# Autodesk Inventor assembly: batterycart assemble
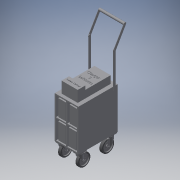
[picture p0: Inventor's stored thumbnail of the model, 180x180]
Saved by Autodesk Inventor 2019 (Build 230136000, 136)
## iProperties
Created: 2018-12-09
Part Number: batterycart assemble
Document SubType Name: Assembly
Designer: Tiberus
Author: Tiberus
## Documents named in this file (7)
- C:\Users\Tiberus\Documents\Inventor\Robotics\batterycart assemble.iam
- C:\Users\Tiberus\Documents\Inventor\Robotics\batter2019.ipt
- C:\Users\Tiberus\Documents\Inventor\Robotics\battery charger 2019.ipt
- C:\Users\Tiberus\Documents\Inventor\Robotics\batterycart skeleton.ipt
- C:\Users\Tiberus\Downloads\AIS2019\2_05456_444.iam
- C:\Users\Tiberus\Documents\Inventor\Robotics\1 battery charger 2019.ipt
- C:\Users\Tiberus\Documents\Inventor\Robotics\cart handle.ipt
## Components (16 placed, 6 different names)
1. batter2019:1 — Mate:7, Mate:8
2. battery charger 2019:1 — Mate:17, Flush:9, Flush:10
3. batterycart skeleton:1 — Mate:1, Mate:2, Mate:3, Mate:4, Mate:5, Mate:6, Mate:7, Mate:8, Mate:9, Mate:10, Mate:11, Mate:12, Mate:13, Mate:14, Mate:15, Mate:16, Mate:17, Mate:18, Mate:19, Mate:20, Mate:21, Flush:1, Flush:2, Flush:3, Flush:4, Flush:5, Flush:6, Flush:7, Flush:8, Flush:9, Flush:10, Mate:22, Flush:11, Flush:12, Mate:23
4. batter2019:2 — Mate:1, Mate:2
5. batter2019:3 — Mate:13, Mate:14
6. batter2019:4 — Mate:10, Mate:16
7. batter2019:5 — Mate:11, Mate:15
8. batter2019:6 — Mate:9, Mate:12
9. batter2019:7 — Mate:5, Mate:6
10. batter2019:8 — Mate:3, Mate:4
11. 2_05456_444:1 [sub-assembly] — Mate:21, Flush:7, Flush:8
12. 2_05456_444:2 [sub-assembly] — Mate:20, Flush:5, Flush:6
13. 2_05456_444:3 [sub-assembly] — Mate:19, Flush:1, Flush:2
14. 2_05456_444:4 [sub-assembly] — Mate:18, Flush:3, Flush:4
15. 1 battery charger 2019:1 — Mate:22, Flush:11, Flush:12
16. cart handle:1 — Mate:23
## Relationships (35: Mate 23, Flush 12)
- Mate:1: batterycart skeleton:1 ↔ batter2019:2
- Mate:2: batterycart skeleton:1 ↔ batter2019:2
- Mate:3: batterycart skeleton:1 ↔ batter2019:8
- Mate:4: batterycart skeleton:1 ↔ batter2019:8
- Mate:5: batterycart skeleton:1 ↔ batter2019:7
- Mate:6: batterycart skeleton:1 ↔ batter2019:7
- Mate:7: batter2019:1 ↔ batterycart skeleton:1
- Mate:8: batter2019:1 ↔ batterycart skeleton:1
- Mate:9: batterycart skeleton:1 ↔ batter2019:6
- Mate:10: batterycart skeleton:1 ↔ batter2019:4
- Mate:11: batterycart skeleton:1 ↔ batter2019:5
- Mate:12: batterycart skeleton:1 ↔ batter2019:6
- Mate:13: batterycart skeleton:1 ↔ batter2019:3
- Mate:14: batterycart skeleton:1 ↔ batter2019:3
- Mate:15: batterycart skeleton:1 ↔ batter2019:5
- Mate:16: batterycart skeleton:1 ↔ batter2019:4
- Mate:17: battery charger 2019:1 ↔ batterycart skeleton:1
- Mate:18: batterycart skeleton:1 ↔ 2_05456_444:4
- Mate:19: batterycart skeleton:1 ↔ 2_05456_444:3
- Mate:20: batterycart skeleton:1 ↔ 2_05456_444:2
- Mate:21: batterycart skeleton:1 ↔ 2_05456_444:1
- Flush:1: batterycart skeleton:1 ↔ 2_05456_444:3
- Flush:2: batterycart skeleton:1 ↔ 2_05456_444:3
- Flush:3: batterycart skeleton:1 ↔ 2_05456_444:4
- Flush:4: batterycart skeleton:1 ↔ 2_05456_444:4
- Flush:5: batterycart skeleton:1 ↔ 2_05456_444:2
- Flush:6: batterycart skeleton:1 ↔ 2_05456_444:2
- Flush:7: batterycart skeleton:1 ↔ 2_05456_444:1
- Flush:8: batterycart skeleton:1 ↔ 2_05456_444:1
- Flush:9 (38.1 mm): battery charger 2019:1 ↔ batterycart skeleton:1
- Flush:10 (31.115 mm): battery charger 2019:1 ↔ batterycart skeleton:1
- Mate:22: batterycart skeleton:1 ↔ 1 battery charger 2019:1
- Flush:11 (31.115 mm): batterycart skeleton:1 ↔ 1 battery charger 2019:1
- Flush:12 (38.1 mm): batterycart skeleton:1 ↔ 1 battery charger 2019:1
- Mate:23: batterycart skeleton:1 ↔ cart handle:1
